# Autodesk Inventor assembly: 4x2 mocowanie
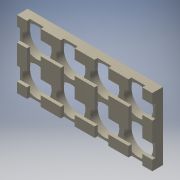
[picture p0: Inventor's stored thumbnail of the model, 180x180]
Saved by Autodesk Inventor 2017 (Build 210142000, 142)
## iProperties
Part Number: 4x2 mocowanie
Material: Ogólny
Document SubType Name: Assembly
Designer: patry
Author: patry
## Documents named in this file (2)
- C:\Users\patry\Desktop\Saper drukowanie\Napinacz\4x2 mocowanie.iam
- C:\Users\patry\Desktop\Saper drukowanie\Napinacz\final cela.ipt
## Components (8 placed, 1 different names)
1. final cela:1 — Zestawiający:1, Równoległy:1, Równoległy:2, Zestawiający:3, Równoległy:5, Równoległy:6
2. final cela:2 — Zestawiający:1, Równoległy:1, Równoległy:2
3. final cela:3 — Zestawiający:7, Zestawiający:8, Równoległy:13
4. final cela:4 — Zestawiający:3, Równoległy:5, Równoległy:6
5. final cela:5
6. final cela:6
7. final cela:7 — Zestawiający:7, Równoległy:13
8. final cela:8 — Zestawiający:8
## Relationships (21: Flush 13, Mate 8)
- Zestawiający:1 [Mate]: final cela:1 ↔ final cela:2
- Równoległy:1 [Flush]: final cela:1 ↔ final cela:2
- Równoległy:2 [Flush]: final cela:1 ↔ final cela:2
- [Mate]: final cela:3 ↔ final cela:4
- [Flush]: final cela:3 ↔ final cela:4
- [Flush]: final cela:3 ↔ final cela:4
- Zestawiający:3 [Mate]: final cela:1 ↔ final cela:4
- Równoległy:5 [Flush]: final cela:1 ↔ final cela:4
- Równoległy:6 [Flush]: final cela:1 ↔ final cela:4
- [Mate]: final cela:5 ↔ final cela:6
- [Flush]: final cela:5 ↔ final cela:6
- [Flush]: final cela:5 ↔ final cela:6
- [Mate]: final cela:7 ↔ final cela:8
- [Flush]: final cela:7 ↔ final cela:8
- [Flush]: final cela:7 ↔ final cela:8
- [Mate]: final cela:5 ↔ final cela:8
- [Flush]: final cela:5 ↔ final cela:8
- [Flush]: final cela:5 ↔ final cela:8
- Zestawiający:7 [Mate]: final cela:3 ↔ final cela:7
- Zestawiający:8 [Mate]: final cela:3 ↔ final cela:8
- Równoległy:13 [Flush]: final cela:3 ↔ final cela:7
## Named parameters: d3_d1 = 0 mm, d4_d2 = 0 mm, d5_d0 = 0 mm, d9_d0 = 0 mm, d10_d1 = 0 mm, d11_d2 = 0 mm, d12_d3_d1 = 0 mm, d13_d4_d2 = 0 mm, d14_d5_d0 = 0 mm, d15_d6 = 0 mm, d16_d7 = 0 mm, d17_d8 = 0 mm
